# Autodesk Inventor assembly: N_core
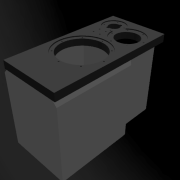
[picture p0: Inventor's stored thumbnail of the model, 180x180]
Saved by Autodesk Inventor 2022 (Build 260153070, 153G)
## iProperties
Created: 2021-11-16
Part Number: N_core
Document SubType Name: Assembly
Designer: kalugin_a
Author: kalugin_a
## Documents named in this file (9)
- C:\Users\kalugin_a\Documents\Inventor\TUTO\N_core.iam
- C:\Users\kalugin_a\Documents\Inventor\TUTO\N_Front.ipt
- C:\Users\kalugin_a\Documents\Inventor\TUTO\N_into_side.ipt
- C:\Users\kalugin_a\Documents\Inventor\TUTO\N-Back_into.ipt
- C:\Users\kalugin_a\Documents\Inventor\TUTO\N_Bottom.ipt
- C:\Users\kalugin_a\Documents\Inventor\TUTO\MID.ipt
- C:\Users\kalugin_a\Documents\Inventor\TUTO\N__side_sticker.ipt
- C:\Users\kalugin_a\Documents\Inventor\TUTO\N__side_sticker_MIR.ipt
- C:\Users\kalugin_a\Documents\Inventor\TUTO\WOOFER.ipt
## Components (10 placed, 9 different names)
1. N_Front:1 — Жесткий:9
2. N_into_side:1 — Заподлицо:2
3. N_into_side:2 — Жесткий:7
4. N-Back_into:1 — Жесткий:3, Жесткий:6, Жесткий:8
5. N_Flane_H — Жесткий:3
6. MID:1
7. N__side_sticker:1 — Заподлицо:2, Жесткий:6
8. N__side_sticker_MIR:1 — Жесткий:7
9. N_Bottom:3 — Жесткий:8, Жесткий:9
10. WOOFER:2
## Relationships (6: WeldJoint 5, Flush 1)
- Заподлицо:2 [Flush]: N_into_side:1 ↔ N__side_sticker:1
- Жесткий:3 [WeldJoint]: N-Back_into:1 ↔ N_Flane_H
- Жесткий:6 [WeldJoint]: N-Back_into:1 ↔ N__side_sticker:1
- Жесткий:7 [WeldJoint]: N_into_side:2 ↔ N__side_sticker_MIR:1
- Жесткий:8 [WeldJoint]: N-Back_into:1 ↔ N_Bottom:3
- Жесткий:9 [WeldJoint]: N_Front:1 ↔ N_Bottom:3
